# Autodesk Inventor assembly: ParallelMecha_V2_BaseFrame_Item40x40
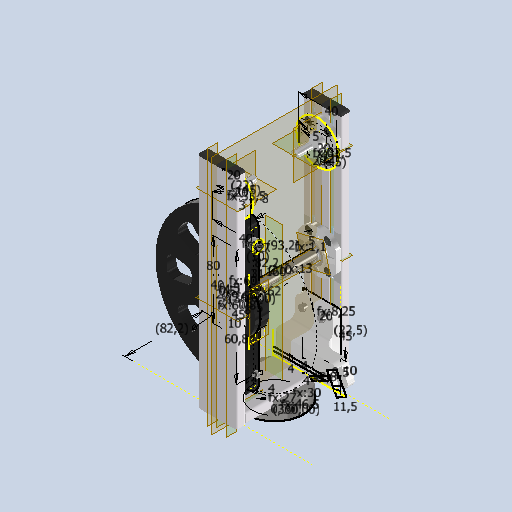
[picture p0: Inventor's stored thumbnail of the model, 512x512]
Saved by Autodesk Inventor 2024 (Build 280153000, 153)
## iProperties
Created: 2022-08-03
Part Number: ParallelMecha_V2_BaseFrame_Item40x40
Document SubType Name: Assembly
Designer: alexw
Mass: 648.14 g
Surface Area: 1074.11 cm^2
Volume: 159.165 cm^3
Author: alexw
## Documents named in this file (24)
- C:\Users\AEWALDER\Documents\Inventor\03_CurrentProjects\MasterThesis\PSM_V1_Rillenkugellager\ParallelMecha_V2_BaseFrame_Item40x40.iam
- C:\Users\AEWALDER\Documents\Inventor\03_CurrentProjects\MasterThesis\PSM_V1_Rillenkugellager\ParallelMecha_DrivenLink_ShaftFixation.ipt
- C:\Users\AEWALDER\Documents\Inventor\03_CurrentProjects\MasterThesis\PSM_V1_Rillenkugellager\ParallelMecha_DrivenShaft.ipt
- C:\Users\AEWALDER\Documents\Inventor\03_CurrentProjects\MasterThesis\PSM_V1_Rillenkugellager\ParallelMecha_Supportlink_BottomShaft.ipt
- C:\Users\AEWALDER\Documents\Inventor\03_CurrentProjects\MasterThesis\PSM_V1_Rillenkugellager\Item\item_0039106_profil_5_40x10_l_150_details_3.ipt
- C:\Users\AEWALDER\Documents\Inventor\03_CurrentProjects\MasterThesis\PSM_V1_Rillenkugellager\Flansch_FemalePart_MainAxis_HeadConnectorBase_V2.1_Item40x40.ipt
- C:\Users\AEWALDER\Documents\Inventor\03_CurrentProjects\MasterThesis\PSM_V1_Rillenkugellager\Item\item_profil_5_40x10_Modified.ipt
- C:\Users\AEWALDER\Documents\Inventor\03_CurrentProjects\MasterThesis\PSM_V1_Rillenkugellager\Item\item_0039114_abdeckkappe_5_40x10_details_3.ipt
- C:\Users\AEWALDER\Documents\Inventor\03_CurrentProjects\MasterThesis\PSM_V1_Rillenkugellager\Item\item_0042510_nutenstein_5_st_m4_details_3.ipt
- C:\Users\AEWALDER\Documents\Inventor\03_CurrentProjects\MasterThesis\PSM_V1_Rillenkugellager\ContentCenter\de-DE\ISO 10642(1)\ISO 10642 - M4 x  16.ipt
- C:\Users\AEWALDER\Documents\Inventor\03_CurrentProjects\MasterThesis\PSM_V1_Rillenkugellager\ContentCenter\de-DE\ISO 10642(1)\ISO 10642 - M4 x  10.ipt
- C:\Users\AEWALDER\Documents\Inventor\03_CurrentProjects\MasterThesis\PSM_V1_Rillenkugellager\SKF_W 61800 R-2RS1.iam
- C:\Users\AEWALDER\Documents\Inventor\03_CurrentProjects\MasterThesis\PSM_V1_Rillenkugellager\circlips_din471_10_1.ipt
- C:\Users\AEWALDER\Documents\Inventor\03_CurrentProjects\MasterThesis\PSM_V1_Rillenkugellager\din_988_10_x_16_x_0_10.ipt
- C:\Users\AEWALDER\Documents\Inventor\03_CurrentProjects\MasterThesis\PSM_V1_Rillenkugellager\Maschinenbauteil\item_0043746_automatik-verbindungssatz_5_details_3.iam
- C:\Users\AEWALDER\Documents\Inventor\03_CurrentProjects\MasterThesis\PSM_V1_Rillenkugellager\ContentCenter\de-DE\ISO 7089\ISO 7089 - 3 - 140 HV(1).ipt
- C:\Users\AEWALDER\Documents\Inventor\03_CurrentProjects\MasterThesis\PSM_V1_Rillenkugellager\ContentCenter\de-DE\ISO 4762(2)\ISO 4762 - M3 x 8ISO.ipt
- C:\Users\AEWALDER\Documents\Inventor\03_CurrentProjects\MasterThesis\PSM_V1_Rillenkugellager\CapstonDisc_ParallelMecha.ipt
- C:\Users\AEWALDER\Documents\Inventor\03_CurrentProjects\MasterThesis\PSM_V1_Rillenkugellager\Axis2_SensorFixatoin.ipt
- C:\Users\AEWALDER\Documents\Inventor\03_CurrentProjects\MasterThesis\PSM_V1_Rillenkugellager\Maschinenbauteil\item_0043746_automatik-verbindungssatz_5_details_3_03.ipt
- C:\Users\AEWALDER\Documents\Inventor\03_CurrentProjects\MasterThesis\PSM_V1_Rillenkugellager\ContentCenter\de-DE\ISO 4762(2)\ISO 4762 - M4 x 12ISO.ipt
- C:\Users\AEWALDER\Documents\Inventor\03_CurrentProjects\MasterThesis\PSM_V1_Rillenkugellager\Capston_Tensioning.ipt
- C:\Users\AEWALDER\Documents\Inventor\03_CurrentProjects\MasterThesis\PSM_V1_Rillenkugellager\ContentCenter\en-US\DIN EN ISO 4032\DIN EN ISO 4032 - M3.ipt
- C:\Users\AEWALDER\Documents\Inventor\03_CurrentProjects\MasterThesis\PSM_V1_Rillenkugellager\ContentCenter\en-US\ISO 4762(1)\DIN EN ISO 4762 - M3 x 16.ipt
## Components (72 placed, 23 different names)
1. Flansch_FemalePart_MainAxis_HeadConnectorBase_V2.1_Item40x40:2 — Passend:59, Passend:60, Tangential:1, Fluchtend:16, Fluchtend:17, Passend:61, Passend:81, Passend:83, Passend:84, Passend:85, Passend:89, Passend:90, Passend:91, Passend:92, Tangential:3, Tangential:4, Tangential:5, Tangential:6
2. ParallelMecha_DrivenLink_ShaftFixation:1 — Passend:70, Passend:93, Passend:94, Passend:95, Passend:96, Passend:115, Passend:116, Passend:117, Passend:118, Passend:128
3. ParallelMecha_DrivenLink_ShaftFixation:2 — Fluchtend:19, Passend:64, Passend:70, Tangential:2, Passend:103, Passend:104, Passend:105, Passend:106, Passend:111, Passend:112, Passend:113, Passend:114
4. SKF_W 61800 R-2RS1:1 [sub-assembly]
5. SKF_W 61800 R-2RS1:2 [sub-assembly] — Passend:132
6. ParallelMecha_DrivenShaft:1 — Passend:126, Passend:130, Passend:131
7. ParallelMecha_Supportlink_BottomShaft:1 — Passend:69, Passend:129, Passend:136, Passend:137, Passend:138, Passend:139, Fluchtend:24, Passend:150, Passend:151, Passend:152, Passend:153, Fluchtend:25
8. ParallelMecha_Supportlink_BottomShaft:2 — Passend:67, Passend:68, Passend:69, Passend:145, Passend:146, Passend:147, Passend:149, Passend:154, Passend:155, Passend:156, Passend:157
9. circlips_din471_10_1:1 — Passend:126
10. circlips_din471_10_1:2 — Passend:130, Passend:133
11. din_988_10_x_16_x_0_10:2
12. item_0039106_profil_5_40x10_l_150_details_3:1 — Fluchtend:22, Fluchtend:23, Passend:76, Passend:79, Passend:80, Winkel:3, Winkel:4, Symmetrie:1, Passend:97, Passend:98, Passend:99, Passend:101, Winkel:7, Winkel:8, Passend:102, Winkel:13, Winkel:14, Passend:121, Passend:122, Passend:128, Passend:129, Passend:134, Passend:135, Winkel:15, Winkel:16, Fluchtend:24, Fluchtend:25, Passend:158, Winkel:21, Passend:159, Fluchtend:26, Passend:160, Fluchtend:28, Passend:174, Winkel:23, Winkel:24, Passend:178, Passend:179
13. item_0039106_profil_5_40x10_l_150_details_3:2 — Passend:56, Fluchtend:10, Fluchtend:11, Fluchtend:19, Passend:64, Passend:67, Passend:68, Tangential:2, Passend:77, Passend:78, Winkel:5, Winkel:6, Symmetrie:1, Winkel:9, Winkel:10, Passend:107, Passend:108, Winkel:11, Winkel:12, Passend:109, Passend:110, Passend:140, Winkel:17, Passend:143, Winkel:18, Winkel:19, Passend:144, Passend:148, Winkel:20, Passend:161, Fluchtend:27, Passend:162, Passend:163
14. item_profil_5_40x10_Modified:1 — Passend:56, Fluchtend:10, Fluchtend:11, Passend:59, Passend:60, Tangential:1, Fluchtend:22, Fluchtend:23, Passend:76, Passend:82, Passend:86, Passend:87, Passend:88, Passend:175
15. item_0039114_abdeckkappe_5_40x10_details_3:1 — Passend:77, Passend:78
16. item_0039114_abdeckkappe_5_40x10_details_3:2 — Passend:79, Passend:80
17. item_0042510_nutenstein_5_st_m4_details_3:1 — Passend:81, Passend:82, Winkel:3
18. item_0042510_nutenstein_5_st_m4_details_3:2 — Passend:83, Winkel:4, Passend:88
19. item_0042510_nutenstein_5_st_m4_details_3:3 — Passend:85, Winkel:6, Passend:86
20. item_0042510_nutenstein_5_st_m4_details_3:4 — Passend:84, Winkel:5, Passend:87
21. ISO 10642 M4x16:1 — Passend:89
22. ISO 10642 M4x16:2 — Passend:90
23. ISO 10642 M4x16:3 — Passend:91
24. ISO 10642 M4x16:4 — Passend:92
25. item_0042510_nutenstein_5_st_m4_details_3:5 — Passend:96, Winkel:8, Passend:102
26. item_0042510_nutenstein_5_st_m4_details_3:6 — Passend:93, Passend:97, Passend:98
27. item_0042510_nutenstein_5_st_m4_details_3:7 — Passend:94, Passend:99
28. item_0042510_nutenstein_5_st_m4_details_3:8 — Passend:95, Passend:101, Winkel:7
29. item_0042510_nutenstein_5_st_m4_details_3:9 — Passend:104, Winkel:9, Passend:108
30. item_0042510_nutenstein_5_st_m4_details_3:10 — Passend:103, Winkel:10, Passend:107
31. item_0042510_nutenstein_5_st_m4_details_3:11 — Passend:105, Winkel:12, Passend:110
32. item_0042510_nutenstein_5_st_m4_details_3:12 — Passend:106, Winkel:11, Passend:109
33. ISO 10642 M4x10:1 — Passend:111
34. ISO 10642 M4x10:2 — Passend:112
35. ISO 10642 M4x10:3 — Passend:113
36. ISO 10642 M4x10:4 — Passend:114
37. ISO 10642 M4x10:5 — Passend:115
38. ISO 10642 M4x10:6 — Passend:116
39. ISO 10642 M4x10:7 — Passend:117
40. ISO 10642 M4x10:8 — Passend:118
41. item_0042510_nutenstein_5_st_m4_details_3:13 — Winkel:13, Passend:121, Passend:138
42. item_0042510_nutenstein_5_st_m4_details_3:14 — Winkel:14, Passend:122, Passend:139
43. din_988_10_x_16_x_0_10:3 — Passend:131, Passend:132, Passend:133
44. item_0042510_nutenstein_5_st_m4_details_3:15 — Passend:134, Winkel:16, Passend:137
45. item_0042510_nutenstein_5_st_m4_details_3:16 — Passend:135, Winkel:15, Passend:136
46. item_0042510_nutenstein_5_st_m4_details_3:17 — Passend:140, Winkel:17, Passend:147
47. item_0042510_nutenstein_5_st_m4_details_3:18 — Passend:148, Winkel:20, Passend:149
48. item_0042510_nutenstein_5_st_m4_details_3:19 — Passend:143, Winkel:18, Passend:146
49. item_0042510_nutenstein_5_st_m4_details_3:20 — Winkel:19, Passend:144, Passend:145
50. CapstonDisc_ParallelMecha:1 — Passend:170, Mate:184, Mate:185, Angle:25, Mate:189
51. ISO 10642 M4x10:9 — Passend:150
52. ISO 10642 M4x10:10 — Passend:151
53. ISO 10642 M4x10:11 — Passend:152
54. ISO 10642 M4x10:12 — Passend:153
55. ISO 10642 M4x10:13 — Passend:154
56. ISO 10642 M4x10:14 — Passend:155
57. ISO 10642 M4x10:15 — Passend:156
58. ISO 10642 M4x10:16 — Passend:157
59. ISO 7089 3:1 — Passend:171
60. ISO 4762 M3 x 8:1 — Passend:170, Passend:171
61. DIN EN ISO 4762 M3 x 16:1 — Mate:190
62. item_0043746_automatik-verbindungssatz_5_details_3:1 [sub-assembly] — Passend:158, Winkel:21, Tangential:3, Passend:159
63. item_0043746_automatik-verbindungssatz_5_details_3:2 [sub-assembly] — Fluchtend:26, Passend:160, Tangential:4
64. item_0043746_automatik-verbindungssatz_5_details_3:3 [sub-assembly] — Passend:161, Passend:162, Tangential:6
65. item_0043746_automatik-verbindungssatz_5_details_3:4 [sub-assembly] — Fluchtend:27, Passend:163, Tangential:5
66. Axis2_SensorFixatoin:1 — Fluchtend:28, Passend:174, Passend:175, Passend:176, Passend:177, Passend:180, Passend:181, Passend:182, Passend:183
67. item_0043746_automatik-verbindungssatz_5_details_3_03:1 — Passend:176, Winkel:23, Passend:178
68. item_0043746_automatik-verbindungssatz_5_details_3_03:2 — Passend:177, Winkel:24, Passend:179
69. ISO 4762 M4 x 12:1 — Passend:180, Passend:181
70. ISO 4762 M4 x 12:2 — Passend:182, Passend:183
71. Capston_Tensioning:1 — Mate:184, Mate:185, Mate:190
72. DIN EN ISO 4032 M3:1 — Angle:25, Mate:189
## Relationships (164: Mate 119, Angle 23, Flush 15, Tangent 6, Symmetry 1)
- [Mate]: ParallelMecha_DrivenLink_ShaftFixation:2 ↔ SKF_W 61800 R-2RS1:1
- [Mate]: ParallelMecha_DrivenLink_ShaftFixation:2 ↔ SKF_W 61800 R-2RS1:1
- [Mate]: ParallelMecha_DrivenLink_ShaftFixation:1 ↔ SKF_W 61800 R-2RS1:2
- [Mate]: ParallelMecha_DrivenLink_ShaftFixation:1 ↔ SKF_W 61800 R-2RS1:2
- [Mate]: SKF_W 61800 R-2RS1:2 ↔ ParallelMecha_DrivenShaft:1
- [Flush]: SKF_W 61800 R-2RS1:1 ↔ ParallelMecha_DrivenShaft:1
- [Mate]: ParallelMecha_DrivenShaft:1 ↔ din_988_10_x_16_x_0_10:2
- [Mate]: SKF_W 61800 R-2RS1:1 ↔ din_988_10_x_16_x_0_10:2
- Passend:56 [Mate]: item_0039106_profil_5_40x10_l_150_details_3:2 ↔ item_profil_5_40x10_Modified:1
- Fluchtend:10 [Flush]: item_0039106_profil_5_40x10_l_150_details_3:2 ↔ item_profil_5_40x10_Modified:1
- Fluchtend:11 [Flush]: item_0039106_profil_5_40x10_l_150_details_3:2 ↔ item_profil_5_40x10_Modified:1
- Passend:59 [Mate]: Flansch_FemalePart_MainAxis_HeadConnectorBase_V2.1_Item40x40:2 ↔ item_profil_5_40x10_Modified:1
- Passend:60 [Mate]: Flansch_FemalePart_MainAxis_HeadConnectorBase_V2.1_Item40x40:2 ↔ item_profil_5_40x10_Modified:1
- Tangential:1: Flansch_FemalePart_MainAxis_HeadConnectorBase_V2.1_Item40x40:2 ↔ item_profil_5_40x10_Modified:1
- Fluchtend:16 [Flush]: Flansch_FemalePart_MainAxis_HeadConnectorBase_V2.1_Item40x40:2
- Fluchtend:17 [Flush]: Flansch_FemalePart_MainAxis_HeadConnectorBase_V2.1_Item40x40:2
- Passend:61 [Mate]: Flansch_FemalePart_MainAxis_HeadConnectorBase_V2.1_Item40x40:2
- [Mate]: SKF_W 61800 R-2RS1:1 ↔ ParallelMecha_DrivenShaft:1
- Fluchtend:19 [Flush]: ParallelMecha_DrivenLink_ShaftFixation:2 ↔ item_0039106_profil_5_40x10_l_150_details_3:2
- Passend:64 [Mate]: ParallelMecha_DrivenLink_ShaftFixation:2 ↔ item_0039106_profil_5_40x10_l_150_details_3:2
- Passend:67 [Mate]: ParallelMecha_Supportlink_BottomShaft:2 ↔ item_0039106_profil_5_40x10_l_150_details_3:2
- Passend:68 [Mate]: ParallelMecha_Supportlink_BottomShaft:2 ↔ item_0039106_profil_5_40x10_l_150_details_3:2
- Passend:69 [Mate]: ParallelMecha_Supportlink_BottomShaft:1 ↔ ParallelMecha_Supportlink_BottomShaft:2
- Passend:70 [Mate]: ParallelMecha_DrivenLink_ShaftFixation:1 ↔ ParallelMecha_DrivenLink_ShaftFixation:2
- Tangential:2: ParallelMecha_DrivenLink_ShaftFixation:2 ↔ item_0039106_profil_5_40x10_l_150_details_3:2
- [Flush]: SKF_W 61800 R-2RS1:2
- [Flush]: SKF_W 61800 R-2RS1:1
- Fluchtend:22 [Flush]: item_0039106_profil_5_40x10_l_150_details_3:1 ↔ item_profil_5_40x10_Modified:1
- Fluchtend:23 [Flush]: item_0039106_profil_5_40x10_l_150_details_3:1 ↔ item_profil_5_40x10_Modified:1
- Passend:76 [Mate]: item_0039106_profil_5_40x10_l_150_details_3:1 ↔ item_profil_5_40x10_Modified:1
- Passend:77 [Mate]: item_0039106_profil_5_40x10_l_150_details_3:2 ↔ item_0039114_abdeckkappe_5_40x10_details_3:1
- Passend:78 [Mate]: item_0039106_profil_5_40x10_l_150_details_3:2 ↔ item_0039114_abdeckkappe_5_40x10_details_3:1
- Passend:79 [Mate]: item_0039106_profil_5_40x10_l_150_details_3:1 ↔ item_0039114_abdeckkappe_5_40x10_details_3:2
- Passend:80 [Mate]: item_0039106_profil_5_40x10_l_150_details_3:1 ↔ item_0039114_abdeckkappe_5_40x10_details_3:2
- Passend:81 [Mate]: Flansch_FemalePart_MainAxis_HeadConnectorBase_V2.1_Item40x40:2 ↔ item_0042510_nutenstein_5_st_m4_details_3:1
- Passend:82 [Mate]: item_profil_5_40x10_Modified:1 ↔ item_0042510_nutenstein_5_st_m4_details_3:1
- Winkel:3 [Angle] (0 deg): item_0039106_profil_5_40x10_l_150_details_3:1 ↔ item_0042510_nutenstein_5_st_m4_details_3:1
- Passend:83 [Mate]: Flansch_FemalePart_MainAxis_HeadConnectorBase_V2.1_Item40x40:2 ↔ item_0042510_nutenstein_5_st_m4_details_3:2
- Passend:84 [Mate]: Flansch_FemalePart_MainAxis_HeadConnectorBase_V2.1_Item40x40:2 ↔ item_0042510_nutenstein_5_st_m4_details_3:4
- Passend:85 [Mate]: Flansch_FemalePart_MainAxis_HeadConnectorBase_V2.1_Item40x40:2 ↔ item_0042510_nutenstein_5_st_m4_details_3:3
- Winkel:4 [Angle] (0 deg): item_0039106_profil_5_40x10_l_150_details_3:1 ↔ item_0042510_nutenstein_5_st_m4_details_3:2
- Winkel:5 [Angle] (0 deg): item_0039106_profil_5_40x10_l_150_details_3:2 ↔ item_0042510_nutenstein_5_st_m4_details_3:4
- Winkel:6 [Angle] (0 deg): item_0039106_profil_5_40x10_l_150_details_3:2 ↔ item_0042510_nutenstein_5_st_m4_details_3:3
- Passend:86 [Mate]: item_profil_5_40x10_Modified:1 ↔ item_0042510_nutenstein_5_st_m4_details_3:3
- Passend:87 [Mate]: item_profil_5_40x10_Modified:1 ↔ item_0042510_nutenstein_5_st_m4_details_3:4
- Passend:88 [Mate]: item_profil_5_40x10_Modified:1 ↔ item_0042510_nutenstein_5_st_m4_details_3:2
- Passend:89 [Mate]: Flansch_FemalePart_MainAxis_HeadConnectorBase_V2.1_Item40x40:2 ↔ ISO 10642 M4x16:1
- Passend:90 [Mate]: Flansch_FemalePart_MainAxis_HeadConnectorBase_V2.1_Item40x40:2 ↔ ISO 10642 M4x16:2
- Passend:91 [Mate]: Flansch_FemalePart_MainAxis_HeadConnectorBase_V2.1_Item40x40:2 ↔ ISO 10642 M4x16:3
- Passend:92 [Mate]: Flansch_FemalePart_MainAxis_HeadConnectorBase_V2.1_Item40x40:2 ↔ ISO 10642 M4x16:4
- Symmetrie:1: item_0039106_profil_5_40x10_l_150_details_3:1 ↔ item_0039106_profil_5_40x10_l_150_details_3:2
- Passend:93 [Mate]: ParallelMecha_DrivenLink_ShaftFixation:1 ↔ item_0042510_nutenstein_5_st_m4_details_3:6
- Passend:94 [Mate]: ParallelMecha_DrivenLink_ShaftFixation:1 ↔ item_0042510_nutenstein_5_st_m4_details_3:7
- Passend:95 [Mate]: ParallelMecha_DrivenLink_ShaftFixation:1 ↔ item_0042510_nutenstein_5_st_m4_details_3:8
- Passend:96 [Mate]: ParallelMecha_DrivenLink_ShaftFixation:1 ↔ item_0042510_nutenstein_5_st_m4_details_3:5
- Passend:97 [Mate]: item_0039106_profil_5_40x10_l_150_details_3:1 ↔ item_0042510_nutenstein_5_st_m4_details_3:6
- Passend:98 [Mate] (0.067 mm): item_0039106_profil_5_40x10_l_150_details_3:1 ↔ item_0042510_nutenstein_5_st_m4_details_3:6
- Passend:99 [Mate]: item_0039106_profil_5_40x10_l_150_details_3:1 ↔ item_0042510_nutenstein_5_st_m4_details_3:7
- Passend:101 [Mate]: item_0039106_profil_5_40x10_l_150_details_3:1 ↔ item_0042510_nutenstein_5_st_m4_details_3:8
- Winkel:7 [Angle] (0 deg): item_0039106_profil_5_40x10_l_150_details_3:1 ↔ item_0042510_nutenstein_5_st_m4_details_3:8
- Winkel:8 [Angle] (0 deg): item_0039106_profil_5_40x10_l_150_details_3:1 ↔ item_0042510_nutenstein_5_st_m4_details_3:5
- Passend:102 [Mate]: item_0039106_profil_5_40x10_l_150_details_3:1 ↔ item_0042510_nutenstein_5_st_m4_details_3:5
- Passend:103 [Mate]: ParallelMecha_DrivenLink_ShaftFixation:2 ↔ item_0042510_nutenstein_5_st_m4_details_3:10
- Passend:104 [Mate]: ParallelMecha_DrivenLink_ShaftFixation:2 ↔ item_0042510_nutenstein_5_st_m4_details_3:9
- Passend:105 [Mate]: ParallelMecha_DrivenLink_ShaftFixation:2 ↔ item_0042510_nutenstein_5_st_m4_details_3:11
- Passend:106 [Mate]: ParallelMecha_DrivenLink_ShaftFixation:2 ↔ item_0042510_nutenstein_5_st_m4_details_3:12
- Winkel:9 [Angle] (0 deg): item_0039106_profil_5_40x10_l_150_details_3:2 ↔ item_0042510_nutenstein_5_st_m4_details_3:9
- Winkel:10 [Angle] (0 deg): item_0039106_profil_5_40x10_l_150_details_3:2 ↔ item_0042510_nutenstein_5_st_m4_details_3:10
- Passend:107 [Mate]: item_0039106_profil_5_40x10_l_150_details_3:2 ↔ item_0042510_nutenstein_5_st_m4_details_3:10
- Passend:108 [Mate]: item_0039106_profil_5_40x10_l_150_details_3:2 ↔ item_0042510_nutenstein_5_st_m4_details_3:9
- Winkel:11 [Angle] (0 deg): item_0039106_profil_5_40x10_l_150_details_3:2 ↔ item_0042510_nutenstein_5_st_m4_details_3:12
- Winkel:12 [Angle] (0 deg): item_0039106_profil_5_40x10_l_150_details_3:2 ↔ item_0042510_nutenstein_5_st_m4_details_3:11
- Passend:109 [Mate]: item_0039106_profil_5_40x10_l_150_details_3:2 ↔ item_0042510_nutenstein_5_st_m4_details_3:12
- Passend:110 [Mate]: item_0039106_profil_5_40x10_l_150_details_3:2 ↔ item_0042510_nutenstein_5_st_m4_details_3:11
- Passend:111 [Mate]: ParallelMecha_DrivenLink_ShaftFixation:2 ↔ ISO 10642 M4x10:1
- Passend:112 [Mate]: ParallelMecha_DrivenLink_ShaftFixation:2 ↔ ISO 10642 M4x10:2
- Passend:113 [Mate]: ParallelMecha_DrivenLink_ShaftFixation:2 ↔ ISO 10642 M4x10:3
- Passend:114 [Mate]: ParallelMecha_DrivenLink_ShaftFixation:2 ↔ ISO 10642 M4x10:4
- Passend:115 [Mate]: ParallelMecha_DrivenLink_ShaftFixation:1 ↔ ISO 10642 M4x10:5
- Passend:116 [Mate]: ParallelMecha_DrivenLink_ShaftFixation:1 ↔ ISO 10642 M4x10:6
- Passend:117 [Mate]: ParallelMecha_DrivenLink_ShaftFixation:1 ↔ ISO 10642 M4x10:7
- Passend:118 [Mate]: ParallelMecha_DrivenLink_ShaftFixation:1 ↔ ISO 10642 M4x10:8
- Winkel:13 [Angle] (0 deg): item_0039106_profil_5_40x10_l_150_details_3:1 ↔ item_0042510_nutenstein_5_st_m4_details_3:13
- Winkel:14 [Angle] (0 deg): item_0039106_profil_5_40x10_l_150_details_3:1 ↔ item_0042510_nutenstein_5_st_m4_details_3:14
- Passend:121 [Mate]: item_0039106_profil_5_40x10_l_150_details_3:1 ↔ item_0042510_nutenstein_5_st_m4_details_3:13
- Passend:122 [Mate]: item_0039106_profil_5_40x10_l_150_details_3:1 ↔ item_0042510_nutenstein_5_st_m4_details_3:14
- Passend:126 [Mate]: ParallelMecha_DrivenShaft:1 ↔ circlips_din471_10_1:1
- [Mate]: circlips_din471_10_1:1 ↔ din_988_10_x_16_x_0_10:2
- Passend:128 [Mate]: ParallelMecha_DrivenLink_ShaftFixation:1 ↔ item_0039106_profil_5_40x10_l_150_details_3:1
- Passend:129 [Mate]: ParallelMecha_Supportlink_BottomShaft:1 ↔ item_0039106_profil_5_40x10_l_150_details_3:1
- Passend:130 [Mate]: ParallelMecha_DrivenShaft:1 ↔ circlips_din471_10_1:2
- Passend:131 [Mate]: ParallelMecha_DrivenShaft:1 ↔ din_988_10_x_16_x_0_10:3
- Passend:132 [Mate]: SKF_W 61800 R-2RS1:2 ↔ din_988_10_x_16_x_0_10:3
- Passend:133 [Mate]: circlips_din471_10_1:2 ↔ din_988_10_x_16_x_0_10:3
- Passend:134 [Mate]: item_0039106_profil_5_40x10_l_150_details_3:1 ↔ item_0042510_nutenstein_5_st_m4_details_3:15
- Passend:135 [Mate]: item_0039106_profil_5_40x10_l_150_details_3:1 ↔ item_0042510_nutenstein_5_st_m4_details_3:16
- Winkel:15 [Angle] (0 deg): item_0039106_profil_5_40x10_l_150_details_3:1 ↔ item_0042510_nutenstein_5_st_m4_details_3:16
- Winkel:16 [Angle] (0 deg): item_0039106_profil_5_40x10_l_150_details_3:1 ↔ item_0042510_nutenstein_5_st_m4_details_3:15
- Passend:136 [Mate]: ParallelMecha_Supportlink_BottomShaft:1 ↔ item_0042510_nutenstein_5_st_m4_details_3:16
- Passend:137 [Mate]: ParallelMecha_Supportlink_BottomShaft:1 ↔ item_0042510_nutenstein_5_st_m4_details_3:15
- Passend:138 [Mate]: ParallelMecha_Supportlink_BottomShaft:1 ↔ item_0042510_nutenstein_5_st_m4_details_3:13
- Passend:139 [Mate]: ParallelMecha_Supportlink_BottomShaft:1 ↔ item_0042510_nutenstein_5_st_m4_details_3:14
- Passend:140 [Mate]: item_0039106_profil_5_40x10_l_150_details_3:2 ↔ item_0042510_nutenstein_5_st_m4_details_3:17
- Winkel:17 [Angle] (0 deg): item_0039106_profil_5_40x10_l_150_details_3:2 ↔ item_0042510_nutenstein_5_st_m4_details_3:17
- Passend:143 [Mate]: item_0039106_profil_5_40x10_l_150_details_3:2 ↔ item_0042510_nutenstein_5_st_m4_details_3:19
- Winkel:18 [Angle] (0 deg): item_0039106_profil_5_40x10_l_150_details_3:2 ↔ item_0042510_nutenstein_5_st_m4_details_3:19
- Winkel:19 [Angle] (0 deg): item_0039106_profil_5_40x10_l_150_details_3:2 ↔ item_0042510_nutenstein_5_st_m4_details_3:20
- Passend:144 [Mate]: item_0039106_profil_5_40x10_l_150_details_3:2 ↔ item_0042510_nutenstein_5_st_m4_details_3:20
- Passend:145 [Mate]: ParallelMecha_Supportlink_BottomShaft:2 ↔ item_0042510_nutenstein_5_st_m4_details_3:20
- Passend:146 [Mate]: ParallelMecha_Supportlink_BottomShaft:2 ↔ item_0042510_nutenstein_5_st_m4_details_3:19
- Passend:147 [Mate]: ParallelMecha_Supportlink_BottomShaft:2 ↔ item_0042510_nutenstein_5_st_m4_details_3:17
- Passend:148 [Mate]: item_0039106_profil_5_40x10_l_150_details_3:2 ↔ item_0042510_nutenstein_5_st_m4_details_3:18
- Winkel:20 [Angle] (0 deg): item_0039106_profil_5_40x10_l_150_details_3:2 ↔ item_0042510_nutenstein_5_st_m4_details_3:18
- Passend:149 [Mate]: ParallelMecha_Supportlink_BottomShaft:2 ↔ item_0042510_nutenstein_5_st_m4_details_3:18
- Fluchtend:24 [Flush]: ParallelMecha_Supportlink_BottomShaft:1 ↔ item_0039106_profil_5_40x10_l_150_details_3:1
- Passend:150 [Mate]: ParallelMecha_Supportlink_BottomShaft:1 ↔ ISO 10642 M4x10:9
- Passend:151 [Mate]: ParallelMecha_Supportlink_BottomShaft:1 ↔ ISO 10642 M4x10:10
- Passend:152 [Mate]: ParallelMecha_Supportlink_BottomShaft:1 ↔ ISO 10642 M4x10:11
- Passend:153 [Mate]: ParallelMecha_Supportlink_BottomShaft:1 ↔ ISO 10642 M4x10:12
- Passend:154 [Mate]: ParallelMecha_Supportlink_BottomShaft:2 ↔ ISO 10642 M4x10:13
- Passend:155 [Mate]: ParallelMecha_Supportlink_BottomShaft:2 ↔ ISO 10642 M4x10:14
- Passend:156 [Mate]: ParallelMecha_Supportlink_BottomShaft:2 ↔ ISO 10642 M4x10:15
- Passend:157 [Mate]: ParallelMecha_Supportlink_BottomShaft:2 ↔ ISO 10642 M4x10:16
- Fluchtend:25 [Flush] (100 mm): ParallelMecha_Supportlink_BottomShaft:1 ↔ item_0039106_profil_5_40x10_l_150_details_3:1
- Passend:158 [Mate]: item_0039106_profil_5_40x10_l_150_details_3:1 ↔ item_0043746_automatik-verbindungssatz_5_details_3:1
- Winkel:21 [Angle] (0 deg): item_0039106_profil_5_40x10_l_150_details_3:1 ↔ item_0043746_automatik-verbindungssatz_5_details_3:1
- Tangential:3: Flansch_FemalePart_MainAxis_HeadConnectorBase_V2.1_Item40x40:2 ↔ item_0043746_automatik-verbindungssatz_5_details_3:1
- Passend:159 [Mate]: item_0039106_profil_5_40x10_l_150_details_3:1 ↔ item_0043746_automatik-verbindungssatz_5_details_3:1
- Fluchtend:26 [Flush]: item_0039106_profil_5_40x10_l_150_details_3:1 ↔ item_0043746_automatik-verbindungssatz_5_details_3:2
- Passend:160 [Mate]: item_0039106_profil_5_40x10_l_150_details_3:1 ↔ item_0043746_automatik-verbindungssatz_5_details_3:2
- Tangential:4: Flansch_FemalePart_MainAxis_HeadConnectorBase_V2.1_Item40x40:2 ↔ item_0043746_automatik-verbindungssatz_5_details_3:2
- Passend:161 [Mate]: item_0039106_profil_5_40x10_l_150_details_3:2 ↔ item_0043746_automatik-verbindungssatz_5_details_3:3
- Fluchtend:27 [Flush]: item_0039106_profil_5_40x10_l_150_details_3:2 ↔ item_0043746_automatik-verbindungssatz_5_details_3:4
- Passend:162 [Mate]: item_0039106_profil_5_40x10_l_150_details_3:2 ↔ item_0043746_automatik-verbindungssatz_5_details_3:3
- Passend:163 [Mate]: item_0039106_profil_5_40x10_l_150_details_3:2 ↔ item_0043746_automatik-verbindungssatz_5_details_3:4
- Tangential:5: Flansch_FemalePart_MainAxis_HeadConnectorBase_V2.1_Item40x40:2 ↔ item_0043746_automatik-verbindungssatz_5_details_3:4
- Tangential:6: Flansch_FemalePart_MainAxis_HeadConnectorBase_V2.1_Item40x40:2 ↔ item_0043746_automatik-verbindungssatz_5_details_3:3
- [Mate]: ISO 7089 3:1 ↔ ISO 4762 M3 x 8:1
- [Mate]: ParallelMecha_DrivenLink_ShaftFixation:2 ↔ CapstonDisc_ParallelMecha:1
- [Mate]: ParallelMecha_DrivenLink_ShaftFixation:2 ↔ CapstonDisc_ParallelMecha:1
- [Angle] (0 deg): ParallelMecha_DrivenLink_ShaftFixation:2 ↔ CapstonDisc_ParallelMecha:1
- [Mate]: CapstonDisc_ParallelMecha:1 ↔ ISO 7089 3:1
- Passend:170 [Mate]: CapstonDisc_ParallelMecha:1 ↔ ISO 4762 M3 x 8:1
- Passend:171 [Mate]: ISO 7089 3:1 ↔ ISO 4762 M3 x 8:1
- Fluchtend:28 [Flush]: item_0039106_profil_5_40x10_l_150_details_3:1 ↔ Axis2_SensorFixatoin:1
- Passend:174 [Mate]: item_0039106_profil_5_40x10_l_150_details_3:1 ↔ Axis2_SensorFixatoin:1
- Passend:175 [Mate]: item_profil_5_40x10_Modified:1 ↔ Axis2_SensorFixatoin:1
- Passend:176 [Mate]: Axis2_SensorFixatoin:1 ↔ item_0043746_automatik-verbindungssatz_5_details_3_03:1
- Passend:177 [Mate]: Axis2_SensorFixatoin:1 ↔ item_0043746_automatik-verbindungssatz_5_details_3_03:2
- Winkel:23 [Angle] (0 deg): item_0039106_profil_5_40x10_l_150_details_3:1 ↔ item_0043746_automatik-verbindungssatz_5_details_3_03:1
- Winkel:24 [Angle] (0 deg): item_0039106_profil_5_40x10_l_150_details_3:1 ↔ item_0043746_automatik-verbindungssatz_5_details_3_03:2
- Passend:178 [Mate]: item_0039106_profil_5_40x10_l_150_details_3:1 ↔ item_0043746_automatik-verbindungssatz_5_details_3_03:1
- Passend:179 [Mate]: item_0039106_profil_5_40x10_l_150_details_3:1 ↔ item_0043746_automatik-verbindungssatz_5_details_3_03:2
- Passend:180 [Mate]: Axis2_SensorFixatoin:1 ↔ ISO 4762 M4 x 12:1
- Passend:181 [Mate]: Axis2_SensorFixatoin:1 ↔ ISO 4762 M4 x 12:1
- Passend:182 [Mate]: Axis2_SensorFixatoin:1 ↔ ISO 4762 M4 x 12:2
- Passend:183 [Mate]: Axis2_SensorFixatoin:1 ↔ ISO 4762 M4 x 12:2
- Mate:184: CapstonDisc_ParallelMecha:1 ↔ Capston_Tensioning:1
- Mate:185: CapstonDisc_ParallelMecha:1 ↔ Capston_Tensioning:1
- [Mate]: DIN EN ISO 4762 M3 x 16:1 ↔ Capston_Tensioning:1
- [Mate]: DIN EN ISO 4762 M3 x 16:1 ↔ DIN EN ISO 4032 M3:1
- Angle:25 (0 deg): CapstonDisc_ParallelMecha:1 ↔ DIN EN ISO 4032 M3:1
- Mate:189: CapstonDisc_ParallelMecha:1 ↔ DIN EN ISO 4032 M3:1
- Mate:190: DIN EN ISO 4762 M3 x 16:1 ↔ Capston_Tensioning:1
